# Autodesk Inventor assembly: camaravision
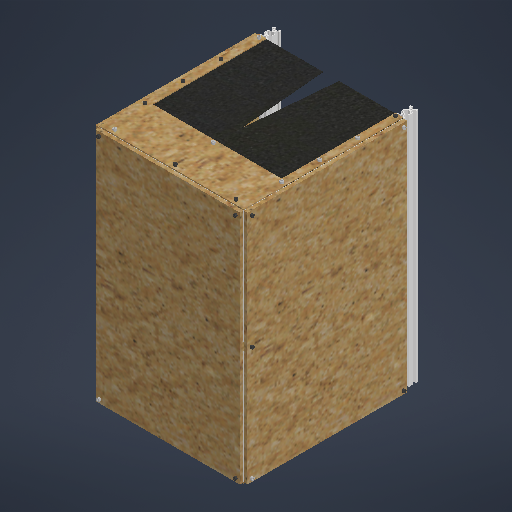
[picture p0: Inventor's stored thumbnail of the model, 512x512]
Saved by Autodesk Inventor 2026.2 (Build 302298010, 298A)
## iProperties
Created: 2026-04-14
Part Number: camaravision
Document SubType Name: Assembly
Designer: grego
Author: grego
## Documents named in this file (13)
- C:\Users\grego\OneDrive\Escritorio\PDM\camaravision.iam
- C:\Users\grego\OneDrive\Escritorio\PDM\VSLOT20x20x340.ipt
- C:\Users\grego\OneDrive\Escritorio\PDM\VSLOT20x40x620.ipt
- C:\Users\grego\OneDrive\Escritorio\PDM\VSLOT20x20x300.ipt
- C:\Users\grego\OneDrive\Escritorio\PDM\VSLOT20x20x400.ipt
- C:\Users\grego\OneDrive\Escritorio\PDM\VSLOT20x20x420.ipt
- C:\Users\grego\OneDrive\Escritorio\PDM\CaraFrontal.ipt
- C:\Users\grego\OneDrive\Escritorio\PDM\CaraMedia.ipt
- C:\Users\grego\OneDrive\Escritorio\PDM\CORNER2028.ipt
- C:\Users\grego\OneDrive\Escritorio\PDM\M5x10.ipt
- C:\Users\grego\OneDrive\Escritorio\PDM\CaraLateral.ipt
- C:\Users\grego\OneDrive\Escritorio\PDM\CaraSuperior.ipt
- C:\Users\grego\OneDrive\Escritorio\PDM\PuertaCuero.ipt
## Components (149 placed, 12 different names)
1. VSLOT20x20x340:1 — Mate:7, Flush:11, Flush:12, Mate:8, Flush:13, Flush:14, Mate:33, Flush:58, Mate:74, Flush:83, Mate:76, Flush:84, Flush:101
2. VSLOT20x40x620:1 — Mate:20, Flush:36, Flush:37, Mate:38, Mate:57, Mate:59, Mate:63
3. VSLOT20x40x620:2 — Mate:28, Mate:41, Mate:45, Mate:47, Flush:70, Mate:61, Flush:94, Flush:95
4. VSLOT20x20x300:1 — Mate:7, Flush:11, Flush:12, Mate:21, Flush:39, Flush:40, Mate:22, Flush:41, Flush:42, Mate:68, Flush:80, Mate:80, Flush:86, Flush:96
5. VSLOT20x20x300:2 — Mate:14, Flush:25, Flush:26, Mate:23, Flush:43, Flush:44, Mate:30, Flush:52, Flush:53, Mate:84, Flush:88, Mate:90, Flush:91, Mate:207, Mate:209
6. VSLOT20x20x300:3 — Mate:8, Flush:13, Flush:14, Mate:27, Mate:31, Flush:54, Flush:55, Mate:50, Flush:71, Mate:66, Flush:79, Mate:208, Flush:100
7. VSLOT20x20x300:4 — Mate:25, Flush:47, Flush:48, Flush:50, Flush:51, Mate:29, Mate:42, Flush:66, Mate:52, Flush:72, Flush:98
8. VSLOT20x20x340:2 — Mate:14, Flush:25, Flush:26, Mate:25, Flush:47, Flush:48, Mate:32, Flush:56, Mate:87, Flush:90, Mate:94, Flush:93, Mate:210
9. VSLOT20x20x340:3 — Mate:24, Flush:45, Flush:46, Mate:26, Flush:49, Mate:37, Flush:62, Mate:78, Flush:85, Mate:81, Flush:87
10. VSLOT20x20x340:4 — Flush:60, Mate:34, Mate:35, Mate:86, Flush:89, Mate:92, Flush:92, Flush:103
11. VSLOT20x20x340:5 — Flush:38, Flush:61, Mate:36, Mate:70, Flush:81, Mate:72, Flush:82, Mate:212, Flush:107
12. VSLOT20x20x400:1 — Mate:20, Flush:36, Flush:37, Flush:38, Mate:21, Flush:39, Flush:40, Mate:64, Flush:78, Mate:67, Mate:69, Mate:73, Flush:97
13. VSLOT20x20x420:1 — Mate:22, Flush:41, Flush:42, Mate:23, Flush:43, Flush:44, Mate:24, Flush:45, Flush:46, Flush:63, Mate:44, Flush:67, Mate:55, Mate:58, Flush:75, Mate:60, Flush:76, Mate:79, Mate:82, Mate:83
14. VSLOT20x20x420:2 — Mate:26, Flush:49, Mate:27, Mate:46, Flush:69, Mate:48, Mate:49, Mate:51, Mate:54, Mate:77, Flush:94, Flush:104
15. VSLOT20x20x400:2 — Mate:28, Flush:50, Flush:51, Mate:29, Mate:40, Flush:65, Mate:43, Mate:85, Mate:88, Flush:102
16. VSLOT20x20x400:3 — Mate:30, Flush:52, Flush:53, Flush:57, Mate:39, Flush:64, Mate:89, Mate:91, Mate:93
17. VSLOT20x20x400:4 — Mate:31, Flush:54, Flush:55, Flush:59, Mate:36, Mate:62, Flush:77, Mate:65, Mate:71, Mate:75, Flush:95, Flush:99, Flush:106
18. CaraFrontal:1 — Mate:32, Flush:56, Flush:57, Flush:60, Mate:34, Mate:35, Mate:213, Mate:214, Mate:215, Mate:216, Mate:217, Mate:218, Mate:219, Mate:220, Mate:221, Mate:222, Mate:223, Mate:224, Mate:225, Mate:226, Mate:227, Mate:228, Mate:229, Mate:230, Mate:231, Mate:232, Mate:233, Mate:234, Mate:235, Mate:236
19. CaraFrontal:2 — Mate:33, Flush:58, Flush:59, Flush:61, Mate:257, Mate:258, Mate:259, Mate:260, Mate:261, Mate:262, Mate:263, Mate:264, Mate:265, Mate:266, Mate:267, Mate:268, Mate:269, Mate:271, Mate:272, Mate:273, Mate:274, Mate:275, Mate:276, Mate:277, Mate:278, Mate:279, Mate:280
20. CaraMedia:1 — Mate:37, Flush:62, Flush:63, Flush:68
21. CORNER2028:1 — Mate:61, Mate:62, Flush:77, Mate:137, Mate:138, Mate:143, Mate:144
22. CORNER2028:2 — Mate:55, Mate:56, Flush:74, Mate:149, Mate:150, Mate:159, Mate:160
23. CORNER2028:3 — Mate:49, Mate:50, Flush:71, Mate:169, Mate:170, Mate:179, Mate:180
24. CORNER2028:4 — Mate:59, Mate:60, Flush:76, Mate:127, Mate:128, Mate:129, Mate:130
25. CORNER2028:5 — Mate:51, Mate:52, Flush:72, Mate:151, Mate:152, Mate:165, Mate:166
26. CORNER2028:6 — Mate:47, Mate:48, Flush:70, Mate:123, Mate:124, Mate:131, Mate:132
27. CORNER2028:7 — Mate:42, Mate:43, Flush:66, Mate:115, Mate:116, Mate:117, Mate:120
28. CORNER2028:8 — Mate:63, Mate:64, Flush:78, Mate:195, Mate:196, Mate:197, Mate:198
29. CORNER2028:9 — Mate:67, Mate:68, Flush:80, Mate:153, Mate:154, Mate:161, Mate:162
30. CORNER2028:10 — Mate:45, Mate:46, Flush:69, Mate:139, Mate:140, Mate:141, Mate:142
31. CORNER2028:11 — Mate:65, Mate:66, Flush:79, Mate:199, Mate:200, Mate:203, Mate:204
32. CORNER2028:12 — Mate:71, Mate:72, Flush:82, Mate:135, Mate:136, Mate:145, Mate:146
33. CORNER2028:13 — Mate:69, Mate:70, Flush:81, Mate:185, Mate:186, Mate:189, Mate:190
34. CORNER2028:14 — Mate:53, Mate:54, Flush:73, Mate:172, Mate:173, Mate:175, Mate:176
35. CORNER2028:15 — Mate:73, Mate:74, Flush:83, Mate:155, Mate:156, Mate:163, Mate:164
36. CORNER2028:16 — Mate:38, Mate:39, Flush:64, Mate:95, Mate:96, Mate:97, Mate:98
37. CORNER2028:17 — Mate:75, Mate:76, Flush:84, Mate:201, Mate:202, Mate:205, Mate:206
38. CORNER2028:18 — Mate:57, Mate:58, Flush:75, Mate:191, Mate:192, Mate:193, Mate:194
39. CORNER2028:19 — Mate:40, Mate:41, Flush:65, Mate:125, Mate:126, Mate:133, Mate:134
40. VSLOT20x20x340:6 — Mate:44, Flush:67, Flush:68, Mate:53, Flush:73, Mate:56, Flush:74, Mate:211, Flush:105
41. CORNER2028:20 — Mate:91, Mate:92, Flush:92, Mate:103, Mate:104, Mate:109, Mate:110
42. CORNER2028:21 — Mate:87, Mate:88, Flush:90, Mate:111, Mate:112, Mate:118, Mate:119
43. CORNER2028:23 — Mate:89, Mate:90, Flush:91, Mate:99, Mate:100, Mate:105, Mate:106
44. CORNER2028:24 — Mate:93, Mate:94, Flush:93, Mate:101, Mate:102, Mate:107, Mate:108
45. CORNER2028:25 — Mate:79, Mate:80, Flush:86, Mate:183, Mate:184, Mate:187, Mate:188
46. CORNER2028:26 — Mate:83, Mate:84, Flush:88, Mate:147, Mate:148, Mate:157, Mate:158
47. CORNER2028:27 — Mate:77, Mate:78, Flush:85, Mate:168, Mate:171, Mate:177, Mate:178
48. CORNER2028:28 — Mate:81, Mate:82, Flush:87, Mate:167, Mate:174, Mate:181, Mate:182
49. CORNER2028:29 — Mate:85, Mate:86, Flush:89, Mate:113, Mate:114, Mate:121, Mate:122
50. M5x10:1 — Mate:95, Mate:96
51. M5x10:2 — Mate:97, Mate:98
52. M5x10:3 — Mate:100, Mate:106
53. M5x10:4 — Mate:102, Mate:107
54. M5x10:5 — Mate:104, Mate:109
55. M5x10:6 — Mate:103, Mate:110
56. M5x10:7 — Mate:101, Mate:108
57. M5x10:8 — Mate:99, Mate:105
58. M5x10:9 — Mate:115, Mate:120
59. M5x10:10 — Mate:114, Mate:121
60. M5x10:11 — Mate:113, Mate:122
61. M5x10:12 — Mate:111, Mate:118
62. M5x10:13 — Mate:112, Mate:119
63. M5x10:14 — Mate:116, Mate:117
64. M5x10:15 — Mate:123, Mate:132
65. M5x10:16 — Mate:127, Mate:130
66. M5x10:17 — Mate:128, Mate:129
67. M5x10:18 — Mate:124, Mate:131
68. M5x10:19 — Mate:125, Mate:133
69. M5x10:20 — Mate:126, Mate:134
70. M5x10:21 — Mate:136, Mate:146
71. M5x10:22 — Mate:138, Mate:144
72. M5x10:23 — Mate:137, Mate:143
73. M5x10:24 — Mate:139, Mate:141
74. M5x10:25 — Mate:135, Mate:145
75. M5x10:26 — Mate:140, Mate:142
76. M5x10:27 — Mate:147, Mate:157
77. M5x10:28 — Mate:148, Mate:158
78. M5x10:29 — Mate:149, Mate:160
79. M5x10:30 — Mate:150, Mate:159
80. M5x10:31 — Mate:151, Mate:165
81. M5x10:32 — Mate:152, Mate:166
82. M5x10:33 — Mate:153, Mate:162
83. M5x10:34 — Mate:154, Mate:161
84. M5x10:35 — Mate:155, Mate:164
85. M5x10:36 — Mate:156, Mate:163
86. M5x10:37 — Mate:167, Mate:182
87. M5x10:38 — Mate:168, Mate:178
88. M5x10:39 — Mate:170, Mate:179
89. M5x10:40 — Mate:171, Mate:177
90. M5x10:41 — Mate:172, Mate:175
91. M5x10:42 — Mate:173, Mate:176
92. M5x10:43 — Mate:174, Mate:181
93. M5x10:44 — Mate:169, Mate:180
94. M5x10:45 — Mate:185, Mate:190
95. M5x10:46 — Mate:186, Mate:189
96. M5x10:47 — Mate:184, Mate:188
97. M5x10:48 — Mate:183, Mate:187
98. M5x10:49 — Mate:191, Mate:193
99. M5x10:50 — Mate:192, Mate:194
100. M5x10:51 — Mate:195, Mate:198
101. M5x10:52 — Mate:196, Mate:197
102. M5x10:53 — Mate:199, Mate:203
103. M5x10:54 — Mate:200, Mate:204
104. M5x10:55 — Mate:201, Mate:206
105. M5x10:56 — Mate:202, Mate:205
106. CaraLateral:1 — Mate:208, Flush:98, Flush:99, Mate:237, Mate:238, Mate:239, Mate:240, Mate:241, Mate:242, Mate:243, Mate:244, Mate:245, Mate:246
107. CaraLateral:2 — Mate:207, Flush:96, Flush:97, Mate:247, Mate:248, Mate:249, Mate:250, Mate:251, Mate:252, Mate:253, Mate:254, Mate:255, Mate:256
108. CaraSuperior:1 — Mate:209, Flush:100, Flush:101, Mate:281, Mate:282, Mate:283, Mate:284, Mate:285, Mate:286, Mate:287, Mate:288
109. PuertaCuero:1 — Mate:210, Flush:102, Flush:103
110. PuertaCuero:2 — Mate:211, Flush:104, Flush:105
111. PuertaCuero:3 — Mate:212, Flush:106, Flush:107, Mate:270
112. M5x10:57 — Mate:214, Mate:229
113. M5x10:58 — Mate:213, Mate:222
114. M5x10:59 — Mate:219, Mate:226
115. M5x10:60 — Mate:216, Mate:223
116. M5x10:61 — Mate:215, Mate:230
117. M5x10:62 — Mate:221, Mate:228
118. M5x10:63 — Mate:220, Mate:227
119. M5x10:64 — Mate:218, Mate:225
120. M5x10:65 — Mate:217, Mate:224
121. M5x10:66 — Mate:231, Mate:236
122. M5x10:67 — Mate:232, Mate:234
123. M5x10:68 — Mate:233, Mate:235
124. M5x10:69 — Mate:237, Mate:242
125. M5x10:70 — Mate:238, Mate:244
126. M5x10:71 — Mate:239, Mate:243
127. M5x10:72 — Mate:240, Mate:246
128. M5x10:73 — Mate:241, Mate:245
129. M5x10:74 — Mate:247, Mate:252
130. M5x10:75 — Mate:248, Mate:253
131. M5x10:76 — Mate:249, Mate:254
132. M5x10:77 — Mate:251, Mate:256
133. M5x10:78 — Mate:250, Mate:255
134. M5x10:79 — Mate:257, Mate:269
135. M5x10:80 — Mate:267, Mate:270
136. M5x10:81 — Mate:263, Mate:275
137. M5x10:82 — Mate:262, Mate:277
138. M5x10:83 — Mate:259, Mate:272
139. M5x10:84 — Mate:258, Mate:278
140. M5x10:85 — Mate:268, Mate:279
141. M5x10:86 — Mate:266, Mate:271
142. M5x10:87 — Mate:265, Mate:280
143. M5x10:88 — Mate:264, Mate:273
144. M5x10:89 — Mate:261, Mate:274
145. M5x10:90 — Mate:260, Mate:276
146. M5x10:91 — Mate:281, Mate:285
147. M5x10:92 — Mate:282, Mate:287
148. M5x10:93 — Mate:283, Mate:288
149. M5x10:94 — Mate:284, Mate:286
## Relationships (350: Mate 272, Flush 78)
- Mate:7: VSLOT20x20x340:1 ↔ VSLOT20x20x300:1
- Flush:11: VSLOT20x20x340:1 ↔ VSLOT20x20x300:1
- Flush:12: VSLOT20x20x340:1 ↔ VSLOT20x20x300:1
- Mate:8: VSLOT20x20x340:1 ↔ VSLOT20x20x300:3
- Flush:13: VSLOT20x20x340:1 ↔ VSLOT20x20x300:3
- Flush:14: VSLOT20x20x340:1 ↔ VSLOT20x20x300:3
- Mate:14: VSLOT20x20x300:2 ↔ VSLOT20x20x340:2
- Flush:25: VSLOT20x20x300:2 ↔ VSLOT20x20x340:2
- Flush:26: VSLOT20x20x300:2 ↔ VSLOT20x20x340:2
- Mate:20: VSLOT20x40x620:1 ↔ VSLOT20x20x400:1
- Flush:36: VSLOT20x40x620:1 ↔ VSLOT20x20x400:1
- Flush:37: VSLOT20x40x620:1 ↔ VSLOT20x20x400:1
- Flush:38: VSLOT20x20x340:5 ↔ VSLOT20x20x400:1
- Mate:21: VSLOT20x20x300:1 ↔ VSLOT20x20x400:1
- Flush:39: VSLOT20x20x300:1 ↔ VSLOT20x20x400:1
- Flush:40: VSLOT20x20x300:1 ↔ VSLOT20x20x400:1
- Mate:22: VSLOT20x20x300:1 ↔ VSLOT20x20x420:1
- Flush:41: VSLOT20x20x300:1 ↔ VSLOT20x20x420:1
- Flush:42: VSLOT20x20x300:1 ↔ VSLOT20x20x420:1
- Mate:23: VSLOT20x20x300:2 ↔ VSLOT20x20x420:1
- Flush:43: VSLOT20x20x300:2 ↔ VSLOT20x20x420:1
- Flush:44: VSLOT20x20x300:2 ↔ VSLOT20x20x420:1
- Mate:24: VSLOT20x20x340:3 ↔ VSLOT20x20x420:1
- Flush:45: VSLOT20x20x340:3 ↔ VSLOT20x20x420:1
- Flush:46: VSLOT20x20x340:3 ↔ VSLOT20x20x420:1
- Mate:25: VSLOT20x20x300:4 ↔ VSLOT20x20x340:2
- Flush:47: VSLOT20x20x300:4 ↔ VSLOT20x20x340:2
- Flush:48: VSLOT20x20x300:4 ↔ VSLOT20x20x340:2
- Mate:26: VSLOT20x20x340:3 ↔ VSLOT20x20x420:2
- Flush:49: VSLOT20x20x340:3 ↔ VSLOT20x20x420:2
- Mate:27: VSLOT20x20x300:3 ↔ VSLOT20x20x420:2
- Mate:28: VSLOT20x40x620:2 ↔ VSLOT20x20x400:2
- Flush:50: VSLOT20x20x300:4 ↔ VSLOT20x20x400:2
- Flush:51: VSLOT20x20x300:4 ↔ VSLOT20x20x400:2
- Mate:29: VSLOT20x20x300:4 ↔ VSLOT20x20x400:2
- Mate:30: VSLOT20x20x300:2 ↔ VSLOT20x20x400:3
- Flush:52: VSLOT20x20x300:2 ↔ VSLOT20x20x400:3
- Flush:53: VSLOT20x20x300:2 ↔ VSLOT20x20x400:3
- Mate:31: VSLOT20x20x300:3 ↔ VSLOT20x20x400:4
- Flush:54: VSLOT20x20x300:3 ↔ VSLOT20x20x400:4
- Flush:55: VSLOT20x20x300:3 ↔ VSLOT20x20x400:4
- Mate:32: VSLOT20x20x340:2 ↔ CaraFrontal:1
- Flush:56: VSLOT20x20x340:2 ↔ CaraFrontal:1
- Flush:57: VSLOT20x20x400:3 ↔ CaraFrontal:1
- Mate:33: VSLOT20x20x340:1 ↔ CaraFrontal:2
- Flush:58: VSLOT20x20x340:1 ↔ CaraFrontal:2
- Flush:59: VSLOT20x20x400:4 ↔ CaraFrontal:2
- Flush:60: VSLOT20x20x340:4 ↔ CaraFrontal:1
- Mate:34: VSLOT20x20x340:4 ↔ CaraFrontal:1
- Mate:35: VSLOT20x20x340:4 ↔ CaraFrontal:1
- Flush:61: VSLOT20x20x340:5 ↔ CaraFrontal:2
- Mate:36: VSLOT20x20x340:5 ↔ VSLOT20x20x400:4
- Mate:37: VSLOT20x20x340:3 ↔ CaraMedia:1
- Flush:62: VSLOT20x20x340:3 ↔ CaraMedia:1
- Flush:63: VSLOT20x20x420:1 ↔ CaraMedia:1
- Mate:38: VSLOT20x40x620:1 ↔ CORNER2028:16
- Mate:39: VSLOT20x20x400:3 ↔ CORNER2028:16
- Flush:64: VSLOT20x20x400:3 ↔ CORNER2028:16
- Mate:40: VSLOT20x20x400:2 ↔ CORNER2028:19
- Mate:41: VSLOT20x40x620:2 ↔ CORNER2028:19
- Flush:65: VSLOT20x20x400:2 ↔ CORNER2028:19
- Mate:42: VSLOT20x20x300:4 ↔ CORNER2028:7
- Mate:43: VSLOT20x20x400:2 ↔ CORNER2028:7
- Flush:66: VSLOT20x20x300:4 ↔ CORNER2028:7
- Mate:44: VSLOT20x20x420:1 ↔ VSLOT20x20x340:6
- Flush:67: VSLOT20x20x420:1 ↔ VSLOT20x20x340:6
- Flush:68: CaraMedia:1 ↔ VSLOT20x20x340:6
- Mate:45: VSLOT20x40x620:2 ↔ CORNER2028:10
- Mate:46: VSLOT20x20x420:2 ↔ CORNER2028:10
- Flush:69: VSLOT20x20x420:2 ↔ CORNER2028:10
- Mate:47: VSLOT20x40x620:2 ↔ CORNER2028:6
- Mate:48: VSLOT20x20x420:2 ↔ CORNER2028:6
- Flush:70: VSLOT20x40x620:2 ↔ CORNER2028:6
- Mate:49: VSLOT20x20x420:2 ↔ CORNER2028:3
- Mate:50: VSLOT20x20x300:3 ↔ CORNER2028:3
- Flush:71: VSLOT20x20x300:3 ↔ CORNER2028:3
- Mate:51: VSLOT20x20x420:2 ↔ CORNER2028:5
- Mate:52: VSLOT20x20x300:4 ↔ CORNER2028:5
- Flush:72: VSLOT20x20x300:4 ↔ CORNER2028:5
- Mate:53: CORNER2028:14 ↔ VSLOT20x20x340:6
- Mate:54: VSLOT20x20x420:2 ↔ CORNER2028:14
- Flush:73: CORNER2028:14 ↔ VSLOT20x20x340:6
- Mate:55: VSLOT20x20x420:1 ↔ CORNER2028:2
- Mate:56: CORNER2028:2 ↔ VSLOT20x20x340:6
- Flush:74: CORNER2028:2 ↔ VSLOT20x20x340:6
- Mate:57: VSLOT20x40x620:1 ↔ CORNER2028:18
- Mate:58: VSLOT20x20x420:1 ↔ CORNER2028:18
- Flush:75: VSLOT20x20x420:1 ↔ CORNER2028:18
- Mate:59: VSLOT20x40x620:1 ↔ CORNER2028:4
- Mate:60: VSLOT20x20x420:1 ↔ CORNER2028:4
- Flush:76: VSLOT20x20x420:1 ↔ CORNER2028:4
- Mate:61: VSLOT20x40x620:2 ↔ CORNER2028:1
- Mate:62: VSLOT20x20x400:4 ↔ CORNER2028:1
- Flush:77: VSLOT20x20x400:4 ↔ CORNER2028:1
- Mate:63: VSLOT20x40x620:1 ↔ CORNER2028:8
- Mate:64: VSLOT20x20x400:1 ↔ CORNER2028:8
- Flush:78: VSLOT20x20x400:1 ↔ CORNER2028:8
- Mate:65: VSLOT20x20x400:4 ↔ CORNER2028:11
- Mate:66: VSLOT20x20x300:3 ↔ CORNER2028:11
- Flush:79: VSLOT20x20x300:3 ↔ CORNER2028:11
- Mate:67: VSLOT20x20x400:1 ↔ CORNER2028:9
- Mate:68: VSLOT20x20x300:1 ↔ CORNER2028:9
- Flush:80: VSLOT20x20x300:1 ↔ CORNER2028:9
- Mate:69: VSLOT20x20x400:1 ↔ CORNER2028:13
- Mate:70: VSLOT20x20x340:5 ↔ CORNER2028:13
- Flush:81: VSLOT20x20x340:5 ↔ CORNER2028:13
- Mate:71: VSLOT20x20x400:4 ↔ CORNER2028:12
- Mate:72: VSLOT20x20x340:5 ↔ CORNER2028:12
- Flush:82: VSLOT20x20x340:5 ↔ CORNER2028:12
- Mate:73: VSLOT20x20x400:1 ↔ CORNER2028:15
- Mate:74: VSLOT20x20x340:1 ↔ CORNER2028:15
- Flush:83: VSLOT20x20x340:1 ↔ CORNER2028:15
- Mate:75: VSLOT20x20x400:4 ↔ CORNER2028:17
- Mate:76: VSLOT20x20x340:1 ↔ CORNER2028:17
- Flush:84: VSLOT20x20x340:1 ↔ CORNER2028:17
- Mate:77: VSLOT20x20x420:2 ↔ CORNER2028:27
- Mate:78: VSLOT20x20x340:3 ↔ CORNER2028:27
- Flush:85: VSLOT20x20x340:3 ↔ CORNER2028:27
- Mate:79: VSLOT20x20x420:1 ↔ CORNER2028:25
- Mate:80: VSLOT20x20x300:1 ↔ CORNER2028:25
- Flush:86: VSLOT20x20x300:1 ↔ CORNER2028:25
- Mate:81: VSLOT20x20x340:3 ↔ CORNER2028:28
- Mate:82: VSLOT20x20x420:1 ↔ CORNER2028:28
- Flush:87: VSLOT20x20x340:3 ↔ CORNER2028:28
- Mate:83: VSLOT20x20x420:1 ↔ CORNER2028:26
- Mate:84: VSLOT20x20x300:2 ↔ CORNER2028:26
- Flush:88: VSLOT20x20x300:2 ↔ CORNER2028:26
- Mate:85: VSLOT20x20x400:2 ↔ CORNER2028:29
- Mate:86: VSLOT20x20x340:4 ↔ CORNER2028:29
- Flush:89: VSLOT20x20x340:4 ↔ CORNER2028:29
- Mate:87: VSLOT20x20x340:2 ↔ CORNER2028:21
- Mate:88: VSLOT20x20x400:2 ↔ CORNER2028:21
- Flush:90: VSLOT20x20x340:2 ↔ CORNER2028:21
- Mate:89: VSLOT20x20x400:3 ↔ CORNER2028:23
- Mate:90: VSLOT20x20x300:2 ↔ CORNER2028:23
- Flush:91: VSLOT20x20x300:2 ↔ CORNER2028:23
- Mate:91: VSLOT20x20x400:3 ↔ CORNER2028:20
- Mate:92: VSLOT20x20x340:4 ↔ CORNER2028:20
- Flush:92: VSLOT20x20x340:4 ↔ CORNER2028:20
- Mate:93: VSLOT20x20x400:3 ↔ CORNER2028:24
- Mate:94: VSLOT20x20x340:2 ↔ CORNER2028:24
- Flush:93: VSLOT20x20x340:2 ↔ CORNER2028:24
- Mate:95: CORNER2028:16 ↔ M5x10:1
- Mate:96: CORNER2028:16 ↔ M5x10:1
- Mate:97: CORNER2028:16 ↔ M5x10:2
- Mate:98: CORNER2028:16 ↔ M5x10:2
- Mate:99: CORNER2028:23 ↔ M5x10:8
- Mate:100: CORNER2028:23 ↔ M5x10:3
- Mate:101: CORNER2028:24 ↔ M5x10:7
- Mate:102: CORNER2028:24 ↔ M5x10:4
- Mate:103: CORNER2028:20 ↔ M5x10:6
- Mate:104: CORNER2028:20 ↔ M5x10:5
- Mate:105: CORNER2028:23 ↔ M5x10:8
- Mate:106: CORNER2028:23 ↔ M5x10:3
- Mate:107: CORNER2028:24 ↔ M5x10:4
- Mate:108: CORNER2028:24 ↔ M5x10:7
- Mate:109: CORNER2028:20 ↔ M5x10:5
- Mate:110: CORNER2028:20 ↔ M5x10:6
- Mate:111: CORNER2028:21 ↔ M5x10:12
- Mate:112: CORNER2028:21 ↔ M5x10:13
- Mate:113: CORNER2028:29 ↔ M5x10:11
- Mate:114: CORNER2028:29 ↔ M5x10:10
- Mate:115: CORNER2028:7 ↔ M5x10:9
- Mate:116: CORNER2028:7 ↔ M5x10:14
- Mate:117: CORNER2028:7 ↔ M5x10:14
- Mate:118: CORNER2028:21 ↔ M5x10:12
- Mate:119: CORNER2028:21 ↔ M5x10:13
- Mate:120: CORNER2028:7 ↔ M5x10:9
- Mate:121: CORNER2028:29 ↔ M5x10:10
- Mate:122: CORNER2028:29 ↔ M5x10:11
- Mate:123: CORNER2028:6 ↔ M5x10:15
- Mate:124: CORNER2028:6 ↔ M5x10:18
- Mate:125: CORNER2028:19 ↔ M5x10:19
- Mate:126: CORNER2028:19 ↔ M5x10:20
- Mate:127: CORNER2028:4 ↔ M5x10:16
- Mate:128: CORNER2028:4 ↔ M5x10:17
- Mate:129: CORNER2028:4 ↔ M5x10:17
- Mate:130: CORNER2028:4 ↔ M5x10:16
- Mate:131: CORNER2028:6 ↔ M5x10:18
- Mate:132: CORNER2028:6 ↔ M5x10:15
- Mate:133: CORNER2028:19 ↔ M5x10:19
- Mate:134: CORNER2028:19 ↔ M5x10:20
- Mate:135: CORNER2028:12 ↔ M5x10:25
- Mate:136: CORNER2028:12 ↔ M5x10:21
- Mate:137: CORNER2028:1 ↔ M5x10:23
- Mate:138: CORNER2028:1 ↔ M5x10:22
- Mate:139: CORNER2028:10 ↔ M5x10:24
- Mate:140: CORNER2028:10 ↔ M5x10:26
- Mate:141: CORNER2028:10 ↔ M5x10:24
- Mate:142: CORNER2028:10 ↔ M5x10:26
- Mate:143: CORNER2028:1 ↔ M5x10:23
- Mate:144: CORNER2028:1 ↔ M5x10:22
- Mate:145: CORNER2028:12 ↔ M5x10:25
- Mate:146: CORNER2028:12 ↔ M5x10:21
- Mate:147: CORNER2028:26 ↔ M5x10:27
- Mate:148: CORNER2028:26 ↔ M5x10:28
- Mate:149: CORNER2028:2 ↔ M5x10:29
- Mate:150: CORNER2028:2 ↔ M5x10:30
- Mate:151: CORNER2028:5 ↔ M5x10:31
- Mate:152: CORNER2028:5 ↔ M5x10:32
- Mate:153: CORNER2028:9 ↔ M5x10:33
- Mate:154: CORNER2028:9 ↔ M5x10:34
- Mate:155: CORNER2028:15 ↔ M5x10:35
- Mate:156: CORNER2028:15 ↔ M5x10:36
- Mate:157: CORNER2028:26 ↔ M5x10:27
- Mate:158: CORNER2028:26 ↔ M5x10:28
- Mate:159: CORNER2028:2 ↔ M5x10:30
- Mate:160: CORNER2028:2 ↔ M5x10:29
- Mate:161: CORNER2028:9 ↔ M5x10:34
- Mate:162: CORNER2028:9 ↔ M5x10:33
- Mate:163: CORNER2028:15 ↔ M5x10:36
- Mate:164: CORNER2028:15 ↔ M5x10:35
- Mate:165: CORNER2028:5 ↔ M5x10:31
- Mate:166: CORNER2028:5 ↔ M5x10:32
- Mate:167: CORNER2028:28 ↔ M5x10:37
- Mate:168: CORNER2028:27 ↔ M5x10:38
- Mate:169: CORNER2028:3 ↔ M5x10:44
- Mate:170: CORNER2028:3 ↔ M5x10:39
- Mate:171: CORNER2028:27 ↔ M5x10:40
- Mate:172: CORNER2028:14 ↔ M5x10:41
- Mate:173: CORNER2028:14 ↔ M5x10:42
- Mate:174: CORNER2028:28 ↔ M5x10:43
- Mate:175: CORNER2028:14 ↔ M5x10:41
- Mate:176: CORNER2028:14 ↔ M5x10:42
- Mate:177: CORNER2028:27 ↔ M5x10:40
- Mate:178: CORNER2028:27 ↔ M5x10:38
- Mate:179: CORNER2028:3 ↔ M5x10:39
- Mate:180: CORNER2028:3 ↔ M5x10:44
- Mate:181: CORNER2028:28 ↔ M5x10:43
- Mate:182: CORNER2028:28 ↔ M5x10:37
- Mate:183: CORNER2028:25 ↔ M5x10:48
- Mate:184: CORNER2028:25 ↔ M5x10:47
- Mate:185: CORNER2028:13 ↔ M5x10:45
- Mate:186: CORNER2028:13 ↔ M5x10:46
- Mate:187: CORNER2028:25 ↔ M5x10:48
- Mate:188: CORNER2028:25 ↔ M5x10:47
- Mate:189: CORNER2028:13 ↔ M5x10:46
- Mate:190: CORNER2028:13 ↔ M5x10:45
- Mate:191: CORNER2028:18 ↔ M5x10:49
- Mate:192: CORNER2028:18 ↔ M5x10:50
- Mate:193: CORNER2028:18 ↔ M5x10:49
- Mate:194: CORNER2028:18 ↔ M5x10:50
- Mate:195: CORNER2028:8 ↔ M5x10:51
- Mate:196: CORNER2028:8 ↔ M5x10:52
- Mate:197: CORNER2028:8 ↔ M5x10:52
- Mate:198: CORNER2028:8 ↔ M5x10:51
- Mate:199: CORNER2028:11 ↔ M5x10:53
- Mate:200: CORNER2028:11 ↔ M5x10:54
- Mate:201: CORNER2028:17 ↔ M5x10:55
- Mate:202: CORNER2028:17 ↔ M5x10:56
- Mate:203: CORNER2028:11 ↔ M5x10:53
- Mate:204: CORNER2028:11 ↔ M5x10:54
- Mate:205: CORNER2028:17 ↔ M5x10:56
- Mate:206: CORNER2028:17 ↔ M5x10:55
- Flush:94: VSLOT20x40x620:2 ↔ VSLOT20x20x420:2
- Flush:95: VSLOT20x40x620:2 ↔ VSLOT20x20x400:4
- Mate:207: VSLOT20x20x300:2 ↔ CaraLateral:2
- Flush:96: VSLOT20x20x300:1 ↔ CaraLateral:2
- Flush:97: VSLOT20x20x400:1 ↔ CaraLateral:2
- Mate:208: VSLOT20x20x300:3 ↔ CaraLateral:1
- Flush:98: VSLOT20x20x300:4 ↔ CaraLateral:1
- Flush:99: VSLOT20x20x400:4 ↔ CaraLateral:1
- Mate:209: VSLOT20x20x300:2 ↔ CaraSuperior:1
- Flush:100: VSLOT20x20x300:3 ↔ CaraSuperior:1
- Flush:101: VSLOT20x20x340:1 ↔ CaraSuperior:1
- Mate:210: VSLOT20x20x340:2 ↔ PuertaCuero:1
- Flush:102: VSLOT20x20x400:2 ↔ PuertaCuero:1
- Flush:103: VSLOT20x20x340:4 ↔ PuertaCuero:1
- Mate:211: VSLOT20x20x340:6 ↔ PuertaCuero:2
- Flush:104: VSLOT20x20x420:2 ↔ PuertaCuero:2
- Flush:105: VSLOT20x20x340:6 ↔ PuertaCuero:2
- Mate:212: VSLOT20x20x340:5 ↔ PuertaCuero:3
- Flush:106: VSLOT20x20x400:4 ↔ PuertaCuero:3
- Flush:107: VSLOT20x20x340:5 ↔ PuertaCuero:3
- Mate:213: CaraFrontal:1 ↔ M5x10:58
- Mate:214: CaraFrontal:1 ↔ M5x10:57
- Mate:215: CaraFrontal:1 ↔ M5x10:61
- Mate:216: CaraFrontal:1 ↔ M5x10:60
- Mate:217: CaraFrontal:1 ↔ M5x10:65
- Mate:218: CaraFrontal:1 ↔ M5x10:64
- Mate:219: CaraFrontal:1 ↔ M5x10:59
- Mate:220: CaraFrontal:1 ↔ M5x10:63
- Mate:221: CaraFrontal:1 ↔ M5x10:62
- Mate:222: CaraFrontal:1 ↔ M5x10:58
- Mate:223: CaraFrontal:1 ↔ M5x10:60
- Mate:224: CaraFrontal:1 ↔ M5x10:65
- Mate:225: CaraFrontal:1 ↔ M5x10:64
- Mate:226: CaraFrontal:1 ↔ M5x10:59
- Mate:227: CaraFrontal:1 ↔ M5x10:63
- Mate:228: CaraFrontal:1 ↔ M5x10:62
- Mate:229: CaraFrontal:1 ↔ M5x10:57
- Mate:230: CaraFrontal:1 ↔ M5x10:61
- Mate:231: CaraFrontal:1 ↔ M5x10:66
- Mate:232: CaraFrontal:1 ↔ M5x10:67
- Mate:233: CaraFrontal:1 ↔ M5x10:68
- Mate:234: CaraFrontal:1 ↔ M5x10:67
- Mate:235: CaraFrontal:1 ↔ M5x10:68
- Mate:236: CaraFrontal:1 ↔ M5x10:66
- Mate:237: CaraLateral:1 ↔ M5x10:69
- Mate:238: CaraLateral:1 ↔ M5x10:70
- Mate:239: CaraLateral:1 ↔ M5x10:71
- Mate:240: CaraLateral:1 ↔ M5x10:72
- Mate:241: CaraLateral:1 ↔ M5x10:73
- Mate:242: CaraLateral:1 ↔ M5x10:69
- Mate:243: CaraLateral:1 ↔ M5x10:71
- Mate:244: CaraLateral:1 ↔ M5x10:70
- Mate:245: CaraLateral:1 ↔ M5x10:73
- Mate:246: CaraLateral:1 ↔ M5x10:72
- Mate:247: CaraLateral:2 ↔ M5x10:74
- Mate:248: CaraLateral:2 ↔ M5x10:75
- Mate:249: CaraLateral:2 ↔ M5x10:76
- Mate:250: CaraLateral:2 ↔ M5x10:78
- Mate:251: CaraLateral:2 ↔ M5x10:77
- Mate:252: CaraLateral:2 ↔ M5x10:74
- Mate:253: CaraLateral:2 ↔ M5x10:75
- Mate:254: CaraLateral:2 ↔ M5x10:76
- Mate:255: CaraLateral:2 ↔ M5x10:78
- Mate:256: CaraLateral:2 ↔ M5x10:77
- Mate:257: CaraFrontal:2 ↔ M5x10:79
- Mate:258: CaraFrontal:2 ↔ M5x10:84
- Mate:259: CaraFrontal:2 ↔ M5x10:83
- Mate:260: CaraFrontal:2 ↔ M5x10:90
- Mate:261: CaraFrontal:2 ↔ M5x10:89
- Mate:262: CaraFrontal:2 ↔ M5x10:82
- Mate:263: CaraFrontal:2 ↔ M5x10:81
- Mate:264: CaraFrontal:2 ↔ M5x10:88
- Mate:265: CaraFrontal:2 ↔ M5x10:87
- Mate:266: CaraFrontal:2 ↔ M5x10:86
- Mate:267: CaraFrontal:2 ↔ M5x10:80
- Mate:268: CaraFrontal:2 ↔ M5x10:85
- Mate:269: CaraFrontal:2 ↔ M5x10:79
- Mate:270: PuertaCuero:3 ↔ M5x10:80
- Mate:271: CaraFrontal:2 ↔ M5x10:86
- Mate:272: CaraFrontal:2 ↔ M5x10:83
- Mate:273: CaraFrontal:2 ↔ M5x10:88
- Mate:274: CaraFrontal:2 ↔ M5x10:89
- Mate:275: CaraFrontal:2 ↔ M5x10:81
- Mate:276: CaraFrontal:2 ↔ M5x10:90
- Mate:277: CaraFrontal:2 ↔ M5x10:82
- Mate:278: CaraFrontal:2 ↔ M5x10:84
- Mate:279: CaraFrontal:2 ↔ M5x10:85
- Mate:280: CaraFrontal:2 ↔ M5x10:87
- Mate:281: CaraSuperior:1 ↔ M5x10:91
- Mate:282: CaraSuperior:1 ↔ M5x10:92
- Mate:283: CaraSuperior:1 ↔ M5x10:93
- Mate:284: CaraSuperior:1 ↔ M5x10:94
- Mate:285: CaraSuperior:1 ↔ M5x10:91
- Mate:286: CaraSuperior:1 ↔ M5x10:94
- Mate:287: CaraSuperior:1 ↔ M5x10:92
- Mate:288: CaraSuperior:1 ↔ M5x10:93
